# Autodesk Inventor assembly: Octave--Black_Keys_Farther_from_White_Keys_and_Closer_to_Actual
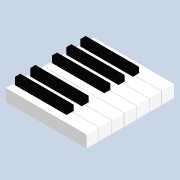
[picture p0: Inventor's stored thumbnail of the model, 180x180]
Saved by Autodesk Inventor 2021 (Build 250183000, 183)
## iProperties
Created: 2021-03-17
Part Number: Octave--Black_Keys_Farther_from_White_Keys_and_Closer_to_Actual
Document SubType Name: Assembly
Designer: Tom
Author: Tom
## Documents named in this file (9)
- C:\Users\Tom\Documents\Inventor\Piano\Octave--Black_Keys_Farther_from_White_Keys_and_Closer_to_Actual.iam
- C:\Users\Tom\Documents\Inventor\Piano\Key--C.ipt
- C:\Users\Tom\Documents\Inventor\Piano\Key--D.ipt
- C:\Users\Tom\Documents\Inventor\Piano\Key--E.ipt
- C:\Users\Tom\Documents\Inventor\Piano\Key--F.ipt
- C:\Users\Tom\Documents\Inventor\Piano\Key--G.ipt
- C:\Users\Tom\Documents\Inventor\Piano\Key--A.ipt
- C:\Users\Tom\Documents\Inventor\Piano\Key--B.ipt
- C:\Users\Tom\Documents\Inventor\Piano\Key--Black.ipt
## Components (12 placed, 8 different names)
1. Key--C:1 — Mate:1, Flush:1, Flush:2, Flush:13
2. Key--D:1 — Mate:1, Flush:1, Flush:2, Mate:2, Flush:3, Flush:4, Mate:7, Flush:14
3. Key--E:1 — Mate:2, Flush:3, Flush:4, Mate:3, Flush:5, Flush:6, Flush:15, Mate:8, Flush:16
4. Key--F:1 — Mate:3, Flush:5, Flush:6, Mate:4, Flush:7, Flush:8
5. Key--G:1 — Mate:4, Flush:7, Flush:8, Mate:5, Flush:9, Flush:10, Mate:9, Flush:17, Flush:18
6. Key--A:1 — Mate:5, Flush:9, Flush:10, Mate:6, Flush:11, Flush:12, Mate:10, Flush:19, Flush:20
7. Key--B:1 — Mate:6, Flush:11, Flush:12, Mate:11, Flush:21, Flush:22
8. Key--Black:1 — Flush:13, Mate:7, Flush:14
9. Key--Black:2 — Flush:15, Mate:8, Flush:16
10. Key--Black:3 — Mate:9, Flush:17, Flush:18
11. Key--Black:4 — Mate:10, Flush:19, Flush:20
12. Key--Black:5 — Mate:11, Flush:21, Flush:22
## Relationships (33: Flush 22, Mate 11)
- Mate:1 (0.7937 mm): Key--C:1 ↔ Key--D:1
- Flush:1: Key--C:1 ↔ Key--D:1
- Flush:2: Key--C:1 ↔ Key--D:1
- Mate:2 (0.7937 mm): Key--D:1 ↔ Key--E:1
- Flush:3: Key--D:1 ↔ Key--E:1
- Flush:4: Key--D:1 ↔ Key--E:1
- Mate:3 (0.7937 mm): Key--E:1 ↔ Key--F:1
- Flush:5: Key--E:1 ↔ Key--F:1
- Flush:6: Key--E:1 ↔ Key--F:1
- Mate:4 (0.7937 mm): Key--F:1 ↔ Key--G:1
- Flush:7: Key--F:1 ↔ Key--G:1
- Flush:8: Key--F:1 ↔ Key--G:1
- Mate:5 (0.7937 mm): Key--G:1 ↔ Key--A:1
- Flush:9: Key--G:1 ↔ Key--A:1
- Flush:10: Key--G:1 ↔ Key--A:1
- Mate:6 (0.7937 mm): Key--A:1 ↔ Key--B:1
- Flush:11: Key--A:1 ↔ Key--B:1
- Flush:12: Key--A:1 ↔ Key--B:1
- Flush:13: Key--C:1 ↔ Key--Black:1
- Mate:7 (1.5875 mm): Key--D:1 ↔ Key--Black:1
- Flush:14: Key--D:1 ↔ Key--Black:1
- Flush:15: Key--E:1 ↔ Key--Black:2
- Mate:8 (1.5875 mm): Key--E:1 ↔ Key--Black:2
- Flush:16: Key--E:1 ↔ Key--Black:2
- Mate:9 (1.5875 mm): Key--G:1 ↔ Key--Black:3
- Flush:17: Key--G:1 ↔ Key--Black:3
- Flush:18: Key--G:1 ↔ Key--Black:3
- Mate:10 (1.5875 mm): Key--A:1 ↔ Key--Black:4
- Flush:19: Key--A:1 ↔ Key--Black:4
- Flush:20: Key--A:1 ↔ Key--Black:4
- Mate:11 (1.5875 mm): Key--B:1 ↔ Key--Black:5
- Flush:21: Key--B:1 ↔ Key--Black:5
- Flush:22: Key--B:1 ↔ Key--Black:5
